# Autodesk Inventor assembly: trackey
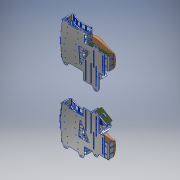
[picture p0: Inventor's stored thumbnail of the model, 180x180]
Saved by Autodesk Inventor 2018 (Build 220112000, 112)
## iProperties
Created: 2018-04-03
Part Number: trackey
Material: 一般
Document SubType Name: Assembly
Designer: NaMACHAN
Mass: 651.315 g
Surface Area: 2801.27 cm^2
Volume: 300.903 cm^3
Density: 2.16453 g/cm^3
Author: NaMACHAN
## Documents named in this file (26)
- C:\Users\NaMACHAN\Dropbox\Project\original\Trackey\inventor\trackey.iam
- C:\Users\NaMACHAN\Dropbox\Project\original\Trackey\inventor\ball.ipt
- C:\Users\NaMACHAN\Dropbox\Project\original\Trackey\inventor\ball_cover.ipt
- C:\Users\NaMACHAN\Dropbox\Project\original\Trackey\inventor\trackball_base.ipt
- C:\Users\NaMACHAN\Dropbox\Project\original\Trackey\inventor\bearing_shaft.ipt
- C:\Users\NaMACHAN\Dropbox\Project\original\Trackey\inventor\bearing.ipt
- C:\Users\NaMACHAN\Dropbox\Project\original\Trackey\inventor\shaft_cover.ipt
- C:\Users\NaMACHAN\Dropbox\Project\original\Trackey\inventor\trackball_spacer.ipt
- C:\Users\NaMACHAN\Dropbox\Project\original\Trackey\inventor\sensor_cover.ipt
- C:\Users\NaMACHAN\Dropbox\Project\original\Trackey\inventor\sensor_sensorcover_spacer.ipt
- C:\Users\NaMACHAN\Dropbox\Project\original\Trackey\inventor\sensor_pcb.ipt
- C:\Users\NaMACHAN\Dropbox\Project\original\Trackey\inventor\trackball_cup.ipt
- C:\Users\NaMACHAN\Dropbox\Project\original\Trackey\inventor\base_plate.ipt
- C:\Users\NaMACHAN\Dropbox\Project\original\Trackey\inventor\key_plate.ipt
- C:\Users\NaMACHAN\Dropbox\Project\original\Trackey\inventor\main_key_cup.ipt
- C:\Users\NaMACHAN\Dropbox\Project\original\Trackey\inventor\palmrest_L_large.ipt
- C:\Users\NaMACHAN\Dropbox\Project\original\Trackey\inventor\palmrest_L_small.ipt
- C:\Users\NaMACHAN\Dropbox\Project\original\Trackey\inventor\palmrest_cup.ipt
- C:\Users\NaMACHAN\Dropbox\Project\original\Trackey\inventor\thumbkey_plate.ipt
- C:\Users\NaMACHAN\Dropbox\Project\original\Trackey\inventor\thumbkey_cup.ipt
- C:\Users\NaMACHAN\Dropbox\Project\original\Trackey\inventor\main_pcb.ipt
- C:\Users\NaMACHAN\Dropbox\Project\original\Trackey\inventor\palmrest_rev3.ipt
- C:\Users\NaMACHAN\Dropbox\Project\original\Trackey\inventor\palmrest_rev3_MIR.ipt
- C:\Users\NaMACHAN\Dropbox\Project\original\Trackey\inventor\main_pcb_spacer.ipt
- C:\Users\NaMACHAN\Dropbox\Project\original\Trackey\inventor\key_plate_col0.ipt
- C:\Users\NaMACHAN\Dropbox\Project\original\Trackey\inventor\main_key_cup_col0.ipt
## Components (67 placed, 25 different names)
1. ball:1 — メイト:17, メイト:147
2. ball_cover:1 — 挿入:7, メイト:20, 挿入:14, メイト:146, メイト:181, フラッシュ:90
3. trackball_base:1 — メイト:1, メイト:2, メイト:3, メイト:4, メイト:5, メイト:6, メイト:7, メイト:8, メイト:9, メイト:13, メイト:14, メイト:15, 挿入:1, メイト:16, メイト:17, メイト:22, メイト:144
4. bearing_shaft:1 — メイト:4, メイト:5, メイト:6, メイト:11
5. bearing_shaft:2 — メイト:7, メイト:8, メイト:9, メイト:10
6. bearing_shaft:3 — メイト:1, メイト:2, メイト:3, メイト:12
7. bearing:1 — メイト:10, メイト:14
8. bearing:2 — メイト:12, メイト:15
9. bearing:3 — メイト:11, メイト:13
10. shaft_cover:1 — 挿入:1, メイト:16, 挿入:2, 挿入:3, 挿入:4, メイト:145, メイト:147
11. trackball_spacer:1 — 挿入:2, メイト:146
12. trackball_spacer:2 — 挿入:3
13. trackball_spacer:3 — 挿入:14, メイト:144, メイト:145
14. trackball_spacer:4 — 挿入:4
15. sensor_cover:1 — 挿入:7, メイト:20, 挿入:8, 挿入:9
16. sensor_sensorcover_spacer:1 — 挿入:8, 挿入:10
17. sensor_sensorcover_spacer:2 — 挿入:9, メイト:21
18. sensor_pcb:1 — 挿入:10, メイト:21
19. trackball_cup:1 — メイト:22, メイト:24, 角度:1, メイト:175, メイト:176, メイト:181, フラッシュ:90
20. base_plate:1 — メイト:24, メイト:53, フラッシュ:26, フラッシュ:49, メイト:103, メイト:128, メイト:129, メイト:130, メイト:131, メイト:132, メイト:133, メイト:134, メイト:135, メイト:136, メイト:137, メイト:140, メイト:141, メイト:142, メイト:143, フラッシュ:77, フラッシュ:79, フラッシュ:82, 角度:1, メイト:175, メイト:176
21. palmrest_L_large:1 — フラッシュ:23, メイト:156, 挿入:24, メイト:167
22. palmrest_L_small:1 — メイト:51, メイト:155, メイト:158, メイト:170
23. palmrest_cup:1 — メイト:51, フラッシュ:23, メイト:53, メイト:168, フラッシュ:79, フラッシュ:82
24. base_plate:2 — フラッシュ:26, メイト:59, メイト:66, メイト:67, メイト:68, メイト:69, メイト:70, メイト:71, メイト:74, メイト:75, メイト:76, メイト:77, メイト:78, メイト:79, メイト:80, メイト:81, メイト:82, メイト:83, フラッシュ:48, フラッシュ:49, メイト:103, フラッシュ:78, フラッシュ:81, メイト:171, メイト:172, 角度:2, 角度:3, メイト:177, メイト:178, メイト:179, メイト:180, メイト:183, メイト:184, メイト:185
25. palmrest_L_large:2 — メイト:148, メイト:153, メイト:164, メイト:166
26. palmrest_L_small:2 — メイト:154, メイト:163, メイト:165
27. palmrest_cup:2 — メイト:59, メイト:148, メイト:169, フラッシュ:78, フラッシュ:81
28. main_key_cup:7 — メイト:66, メイト:74, メイト:81, フラッシュ:43, フラッシュ:48, メイト:114, メイト:115, フラッシュ:65
29. main_key_cup:8 — メイト:67, メイト:68, メイト:77, メイト:78, フラッシュ:45, フラッシュ:46, メイト:108, フラッシュ:62, メイト:109
30. main_key_cup:9 — メイト:69, メイト:79, メイト:80, フラッシュ:46, メイト:106, フラッシュ:61, メイト:107, フラッシュ:93
31. main_key_cup:10 — メイト:70, メイト:75, メイト:76, フラッシュ:44, フラッシュ:45, メイト:110, メイト:111, フラッシュ:63
32. main_key_cup:11 — メイト:71, メイト:82, メイト:83, フラッシュ:43, フラッシュ:44, メイト:112, フラッシュ:64, メイト:113
33. thumbkey_plate:1 — メイト:173, フラッシュ:88, フラッシュ:89
34. thumbkey_plate:2 — メイト:174, フラッシュ:86, フラッシュ:87
35. key_plate:9 — メイト:106, フラッシュ:61, メイト:107
36. key_plate:10 — メイト:108, フラッシュ:62, メイト:109
37. key_plate:11 — メイト:110, メイト:111, フラッシュ:63
38. key_plate:13 — メイト:114, メイト:115, フラッシュ:65
39. key_plate:14 — メイト:112, フラッシュ:64, メイト:113
40. main_key_cup:13 — メイト:135, メイト:141
41. main_key_cup:14 — メイト:133, メイト:142, フラッシュ:77
42. main_key_cup:15 — メイト:134, メイト:136, メイト:137
43. main_key_cup:16 — メイト:132, メイト:143
44. main_key_cup:17 — メイト:131, メイト:140
45. main_key_cup:18 — メイト:128, メイト:129, メイト:130
46. key_plate:15
47. key_plate:16
48. key_plate:17
49. key_plate:18
50. key_plate:19
51. key_plate:20
52. palmrest_rev3:1 — メイト:153, メイト:154, メイト:161, メイト:166, メイト:169
53. palmrest_rev3_MIR:1 — メイト:155, メイト:156, メイト:158, メイト:162, メイト:167, メイト:168, メイト:170
54. main_pcb_spacer:1 — 挿入:15, メイト:163, メイト:165
55. main_pcb:1 — 挿入:15, 挿入:16, 挿入:17, 挿入:18
56. main_pcb_spacer:2 — 挿入:17, メイト:161
57. main_pcb_spacer:3 — 挿入:16
58. main_pcb_spacer:4 — 挿入:18, メイト:164
59. main_pcb:2 — 挿入:20, 挿入:21, 挿入:22, 挿入:23
60. main_pcb_spacer:5 — 挿入:20, メイト:162
61. main_pcb_spacer:6 — 挿入:23, 挿入:24
62. main_pcb_spacer:7 — 挿入:22
63. main_pcb_spacer:8 — 挿入:21
64. thumbkey_cup:2 — メイト:171, メイト:174, フラッシュ:86, フラッシュ:87, 角度:3, メイト:178, メイト:179
65. thumbkey_cup:3 — メイト:172, メイト:173, フラッシュ:88, フラッシュ:89, 角度:2, メイト:177, メイト:180
66. key_plate_col0:1 — フラッシュ:91, フラッシュ:92, メイト:182
67. main_key_cup_col0:1 — フラッシュ:91, フラッシュ:92, メイト:182, メイト:183, メイト:184, メイト:185, フラッシュ:93
## Relationships (172: Mate 113, Flush 38, Insert 18, Angle 3)
- メイト:1 [Mate] (1.5 mm): trackball_base:1 ↔ bearing_shaft:3
- メイト:2 [Mate] (1.5 mm): trackball_base:1 ↔ bearing_shaft:3
- メイト:3 [Mate]: trackball_base:1 ↔ bearing_shaft:3
- メイト:4 [Mate] (1.5 mm): trackball_base:1 ↔ bearing_shaft:1
- メイト:5 [Mate] (1.5 mm): trackball_base:1 ↔ bearing_shaft:1
- メイト:6 [Mate]: trackball_base:1 ↔ bearing_shaft:1
- メイト:7 [Mate] (1.5 mm): trackball_base:1 ↔ bearing_shaft:2
- メイト:8 [Mate] (1.5 mm): trackball_base:1 ↔ bearing_shaft:2
- メイト:9 [Mate]: trackball_base:1 ↔ bearing_shaft:2
- メイト:10 [Mate]: bearing_shaft:2 ↔ bearing:1
- メイト:11 [Mate]: bearing_shaft:1 ↔ bearing:3
- メイト:12 [Mate]: bearing_shaft:3 ↔ bearing:2
- メイト:13 [Mate] (1 mm): trackball_base:1 ↔ bearing:3
- メイト:14 [Mate] (1 mm): trackball_base:1 ↔ bearing:1
- メイト:15 [Mate] (1 mm): trackball_base:1 ↔ bearing:2
- 挿入:1 [Insert]: trackball_base:1 ↔ shaft_cover:1
- メイト:16 [Mate]: trackball_base:1 ↔ shaft_cover:1
- メイト:17 [Mate]: ball:1 ↔ trackball_base:1
- 挿入:2 [Insert]: shaft_cover:1 ↔ trackball_spacer:1
- 挿入:3 [Insert]: shaft_cover:1 ↔ trackball_spacer:2
- 挿入:4 [Insert]: shaft_cover:1 ↔ trackball_spacer:4
- 挿入:7 [Insert]: ball_cover:1 ↔ sensor_cover:1
- メイト:20 [Mate]: ball_cover:1 ↔ sensor_cover:1
- 挿入:8 [Insert]: sensor_cover:1 ↔ sensor_sensorcover_spacer:1
- 挿入:9 [Insert]: sensor_cover:1 ↔ sensor_sensorcover_spacer:2
- 挿入:10 [Insert]: sensor_sensorcover_spacer:1 ↔ sensor_pcb:1
- メイト:21 [Mate]: sensor_sensorcover_spacer:2 ↔ sensor_pcb:1
- メイト:22 [Mate] (10 mm): trackball_base:1 ↔ trackball_cup:1
- メイト:24 [Mate]: trackball_cup:1 ↔ base_plate:1
- メイト:51 [Mate]: palmrest_L_small:1 ↔ palmrest_cup:1
- フラッシュ:23 [Flush] (-5 mm): palmrest_L_large:1 ↔ palmrest_cup:1
- メイト:53 [Mate]: base_plate:1 ↔ palmrest_cup:1
- フラッシュ:26 [Flush]: base_plate:1 ↔ base_plate:2
- [Mate]: palmrest_L_small:2 ↔ palmrest_cup:2
- [Flush] (-5 mm): palmrest_L_large:2 ↔ palmrest_cup:2
- メイト:59 [Mate]: base_plate:2 ↔ palmrest_cup:2
- メイト:66 [Mate]: base_plate:2 ↔ main_key_cup:7
- メイト:67 [Mate]: base_plate:2 ↔ main_key_cup:8
- メイト:68 [Mate]: base_plate:2 ↔ main_key_cup:8
- メイト:69 [Mate]: base_plate:2 ↔ main_key_cup:9
- メイト:70 [Mate]: base_plate:2 ↔ main_key_cup:10
- メイト:71 [Mate]: base_plate:2 ↔ main_key_cup:11
- メイト:74 [Mate] (1 mm): base_plate:2 ↔ main_key_cup:7
- メイト:75 [Mate] (1 mm): base_plate:2 ↔ main_key_cup:10
- メイト:76 [Mate] (1 mm): base_plate:2 ↔ main_key_cup:10
- メイト:77 [Mate] (1 mm): base_plate:2 ↔ main_key_cup:8
- メイト:78 [Mate] (1 mm): base_plate:2 ↔ main_key_cup:8
- メイト:79 [Mate] (1 mm): base_plate:2 ↔ main_key_cup:9
- メイト:80 [Mate] (1 mm): base_plate:2 ↔ main_key_cup:9
- メイト:81 [Mate] (1 mm): base_plate:2 ↔ main_key_cup:7
- メイト:82 [Mate] (1 mm): base_plate:2 ↔ main_key_cup:11
- メイト:83 [Mate] (1 mm): base_plate:2 ↔ main_key_cup:11
- フラッシュ:43 [Flush]: main_key_cup:7 ↔ main_key_cup:11
- フラッシュ:44 [Flush] (5 mm): main_key_cup:10 ↔ main_key_cup:11
- フラッシュ:45 [Flush] (2 mm): main_key_cup:8 ↔ main_key_cup:10
- フラッシュ:46 [Flush] (3 mm): main_key_cup:8 ↔ main_key_cup:9
- フラッシュ:48 [Flush] (-3 mm): base_plate:2 ↔ main_key_cup:7
- フラッシュ:49 [Flush]: base_plate:1 ↔ base_plate:2
- メイト:103 [Mate] (150 mm): base_plate:1 ↔ base_plate:2
- メイト:106 [Mate]: main_key_cup:9 ↔ key_plate:9
- フラッシュ:61 [Flush]: main_key_cup:9 ↔ key_plate:9
- メイト:107 [Mate] (6 mm): main_key_cup:9 ↔ key_plate:9
- メイト:108 [Mate]: main_key_cup:8 ↔ key_plate:10
- フラッシュ:62 [Flush]: main_key_cup:8 ↔ key_plate:10
- メイト:109 [Mate] (3 mm): main_key_cup:8 ↔ key_plate:10
- メイト:110 [Mate] (5 mm): main_key_cup:10 ↔ key_plate:11
- メイト:111 [Mate]: main_key_cup:10 ↔ key_plate:11
- フラッシュ:63 [Flush]: main_key_cup:10 ↔ key_plate:11
- メイト:112 [Mate]: main_key_cup:11 ↔ key_plate:14
- フラッシュ:64 [Flush]: main_key_cup:11 ↔ key_plate:14
- メイト:113 [Mate] (10 mm): main_key_cup:11 ↔ key_plate:14
- メイト:114 [Mate] (13 mm): main_key_cup:7 ↔ key_plate:13
- メイト:115 [Mate]: main_key_cup:7 ↔ key_plate:13
- フラッシュ:65 [Flush]: main_key_cup:7 ↔ key_plate:13
- [Flush]: main_key_cup:13 ↔ main_key_cup:17
- [Flush] (5 mm): main_key_cup:16 ↔ main_key_cup:17
- [Flush] (2 mm): main_key_cup:14 ↔ main_key_cup:16
- [Flush] (3 mm): main_key_cup:14 ↔ main_key_cup:15
- [Flush] (2 mm): main_key_cup:15 ↔ main_key_cup:18
- [Flush]: main_key_cup:18 ↔ key_plate:15
- [Mate] (9 mm): main_key_cup:18 ↔ key_plate:15
- [Mate]: main_key_cup:18 ↔ key_plate:15
- [Mate]: main_key_cup:15 ↔ key_plate:16
- [Flush]: main_key_cup:15 ↔ key_plate:16
- [Mate] (6 mm): main_key_cup:15 ↔ key_plate:16
- [Mate]: main_key_cup:14 ↔ key_plate:17
- [Flush]: main_key_cup:14 ↔ key_plate:17
- [Mate] (3 mm): main_key_cup:14 ↔ key_plate:17
- [Mate] (5 mm): main_key_cup:16 ↔ key_plate:18
- [Mate]: main_key_cup:16 ↔ key_plate:18
- [Flush]: main_key_cup:16 ↔ key_plate:18
- [Mate]: main_key_cup:17 ↔ key_plate:20
- [Flush]: main_key_cup:17 ↔ key_plate:20
- [Mate] (10 mm): main_key_cup:17 ↔ key_plate:20
- [Mate] (13 mm): main_key_cup:13 ↔ key_plate:19
- [Mate]: main_key_cup:13 ↔ key_plate:19
- [Flush]: main_key_cup:13 ↔ key_plate:19
- メイト:128 [Mate] (2 mm): base_plate:1 ↔ main_key_cup:18
- メイト:129 [Mate] (2 mm): base_plate:1 ↔ main_key_cup:18
- メイト:130 [Mate]: base_plate:1 ↔ main_key_cup:18
- メイト:131 [Mate]: base_plate:1 ↔ main_key_cup:17
- メイト:132 [Mate]: base_plate:1 ↔ main_key_cup:16
- メイト:133 [Mate]: base_plate:1 ↔ main_key_cup:14
- メイト:134 [Mate]: base_plate:1 ↔ main_key_cup:15
- メイト:135 [Mate]: base_plate:1 ↔ main_key_cup:13
- メイト:136 [Mate] (2 mm): base_plate:1 ↔ main_key_cup:15
- メイト:137 [Mate] (2 mm): base_plate:1 ↔ main_key_cup:15
- メイト:140 [Mate] (2 mm): base_plate:1 ↔ main_key_cup:17
- メイト:141 [Mate] (2 mm): base_plate:1 ↔ main_key_cup:13
- メイト:142 [Mate] (2 mm): base_plate:1 ↔ main_key_cup:14
- メイト:143 [Mate] (2 mm): base_plate:1 ↔ main_key_cup:16
- フラッシュ:77 [Flush] (-10 mm): base_plate:1 ↔ main_key_cup:14
- 挿入:14 [Insert]: ball_cover:1 ↔ trackball_spacer:3
- メイト:144 [Mate]: trackball_base:1 ↔ trackball_spacer:3
- メイト:145 [Mate]: shaft_cover:1 ↔ trackball_spacer:3
- メイト:146 [Mate]: ball_cover:1 ↔ trackball_spacer:1
- メイト:147 [Mate] (8 mm): ball:1 ↔ shaft_cover:1
- メイト:148 [Mate]: palmrest_L_large:2 ↔ palmrest_cup:2
- メイト:153 [Mate]: palmrest_L_large:2 ↔ palmrest_rev3:1
- メイト:154 [Mate]: palmrest_L_small:2 ↔ palmrest_rev3:1
- メイト:155 [Mate]: palmrest_L_small:1 ↔ palmrest_rev3_MIR:1
- メイト:156 [Mate]: palmrest_L_large:1 ↔ palmrest_rev3_MIR:1
- メイト:158 [Mate]: palmrest_L_small:1 ↔ palmrest_rev3_MIR:1
- 挿入:15 [Insert]: main_pcb_spacer:1 ↔ main_pcb:1
- 挿入:16 [Insert]: main_pcb:1 ↔ main_pcb_spacer:3
- 挿入:17 [Insert]: main_pcb:1 ↔ main_pcb_spacer:2
- 挿入:18 [Insert]: main_pcb:1 ↔ main_pcb_spacer:4
- メイト:161 [Mate]: palmrest_rev3:1 ↔ main_pcb_spacer:2
- 挿入:20 [Insert]: main_pcb:2 ↔ main_pcb_spacer:5
- 挿入:21 [Insert]: main_pcb:2 ↔ main_pcb_spacer:8
- 挿入:22 [Insert]: main_pcb:2 ↔ main_pcb_spacer:7
- 挿入:23 [Insert]: main_pcb:2 ↔ main_pcb_spacer:6
- 挿入:24 [Insert]: palmrest_L_large:1 ↔ main_pcb_spacer:6
- メイト:162 [Mate]: palmrest_rev3_MIR:1 ↔ main_pcb_spacer:5
- メイト:163 [Mate]: palmrest_L_small:2 ↔ main_pcb_spacer:1
- メイト:164 [Mate]: palmrest_L_large:2 ↔ main_pcb_spacer:4
- メイト:165 [Mate]: palmrest_L_small:2 ↔ main_pcb_spacer:1
- メイト:166 [Mate]: palmrest_L_large:2 ↔ palmrest_rev3:1
- メイト:167 [Mate]: palmrest_L_large:1 ↔ palmrest_rev3_MIR:1
- メイト:168 [Mate]: palmrest_cup:1 ↔ palmrest_rev3_MIR:1
- メイト:169 [Mate]: palmrest_cup:2 ↔ palmrest_rev3:1
- メイト:170 [Mate]: palmrest_L_small:1 ↔ palmrest_rev3_MIR:1
- フラッシュ:78 [Flush] (-15 mm): base_plate:2 ↔ palmrest_cup:2
- フラッシュ:79 [Flush] (-15 mm): base_plate:1 ↔ palmrest_cup:1
- フラッシュ:81 [Flush]: base_plate:2 ↔ palmrest_cup:2
- フラッシュ:82 [Flush]: base_plate:1 ↔ palmrest_cup:1
- メイト:171 [Mate]: base_plate:2 ↔ thumbkey_cup:2
- メイト:172 [Mate]: base_plate:2 ↔ thumbkey_cup:3
- メイト:173 [Mate]: thumbkey_plate:1 ↔ thumbkey_cup:3
- メイト:174 [Mate]: thumbkey_plate:2 ↔ thumbkey_cup:2
- フラッシュ:86 [Flush]: thumbkey_plate:2 ↔ thumbkey_cup:2
- フラッシュ:87 [Flush] (5 mm): thumbkey_plate:2 ↔ thumbkey_cup:2
- フラッシュ:88 [Flush] (-5 mm): thumbkey_plate:1 ↔ thumbkey_cup:3
- フラッシュ:89 [Flush]: thumbkey_plate:1 ↔ thumbkey_cup:3
- 角度:1 [Angle] (60 deg): trackball_cup:1 ↔ base_plate:1
- メイト:175 [Mate] (3 mm): trackball_cup:1 ↔ base_plate:1
- メイト:176 [Mate] (-40 mm): trackball_cup:1 ↔ base_plate:1
- 角度:2 [Angle] (30 deg): base_plate:2 ↔ thumbkey_cup:3
- 角度:3 [Angle] (30 deg): base_plate:2 ↔ thumbkey_cup:2
- メイト:177 [Mate] (-20 mm): base_plate:2 ↔ thumbkey_cup:3
- メイト:178 [Mate] (-35 mm): base_plate:2 ↔ thumbkey_cup:2
- メイト:179 [Mate] (-7 mm): base_plate:2 ↔ thumbkey_cup:2
- メイト:180 [Mate] (-20 mm): base_plate:2 ↔ thumbkey_cup:3
- メイト:181 [Mate]: ball_cover:1 ↔ trackball_cup:1
- フラッシュ:90 [Flush]: ball_cover:1 ↔ trackball_cup:1
- フラッシュ:91 [Flush]: key_plate_col0:1 ↔ main_key_cup_col0:1
- フラッシュ:92 [Flush] (-3 mm): key_plate_col0:1 ↔ main_key_cup_col0:1
- メイト:182 [Mate]: key_plate_col0:1 ↔ main_key_cup_col0:1
- メイト:183 [Mate]: base_plate:2 ↔ main_key_cup_col0:1
- メイト:184 [Mate] (1.5 mm): base_plate:2 ↔ main_key_cup_col0:1
- メイト:185 [Mate] (1.5 mm): base_plate:2 ↔ main_key_cup_col0:1
- フラッシュ:93 [Flush] (2 mm): main_key_cup:9 ↔ main_key_cup_col0:1
## Named parameters: d403_d390 = 0 mm, d404_d391 = -5 mm, d521_d509 = 0 mm, d522_d510 = 0 mm, d523_d511 = 3 mm, d524_d512 = 5 mm, d525_d513 = 0 mm, d526_d514 = 0 mm, d527_d515 = 0 mm, d528_d516 = 0 mm, d529_d517 = 10 mm, d530_d518 = 13 mm, d531_d519 = 0 mm, d532_d520 = 0 mm, d533_d503 = 0 mm, d534_d504 = 9 mm, d535_d505 = 0 mm, d536_d506 = 0 mm, d537_d507 = 0 mm, d538_d508 = 6 mm, d539_d451 = 0 mm, d540_d452 = 5 mm, d541_d453 = 2 mm, d542_d454 = 3 mm, d543_d455 = 2 mm
